# Autodesk Inventor assembly: Door 2
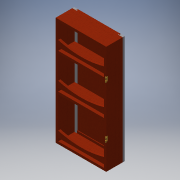
[picture p0: Inventor's stored thumbnail of the model, 180x180]
Saved by Autodesk Inventor 2016 (Build 200138000, 138)
## iProperties
Created: 2017-10-31
Part Number: Door 2
Document SubType Name: Assembly
Designer: mathaetaes
Author: mathaetaes
## Documents named in this file (7)
- E:\Projects\3D Printer\printer projects\My Designs\Bar Cabinet 2.20.2018\Door 2.iam
- E:\Projects\3D Printer\printer projects\My Designs\Bar Cabinet 2.20.2018\Door top.ipt
- E:\Projects\3D Printer\printer projects\My Designs\Bar Cabinet 2.20.2018\Door retention wall.ipt
- E:\Projects\3D Printer\printer projects\My Designs\Bar Cabinet 2.20.2018\Door Shelf.ipt
- E:\Projects\3D Printer\printer projects\My Designs\Bar Cabinet 2.20.2018\Door 2 Side.ipt
- E:\Projects\3D Printer\printer projects\My Designs\Bar Cabinet 2.20.2018\Door Moulding Assembled.iam
- E:\Projects\3D Printer\printer projects\My Designs\Bar Cabinet 2.20.2018\hinge left.ipt
## Components (12 placed, 6 different names)
1. Door top:1 — Flush:21, Flush:22, Mate:32, Flush:30, Flush:31, Mate:33, Flush:33
2. Door retention wall:1 — Mate:20, Flush:20, Mate:34
3. Door Shelf:1 — Mate:10, Mate:12, Mate:15, Flush:15, Flush:16, Mate:19
4. Door retention wall:2 — Mate:10, Flush:14, Mate:16
5. Door 2 Side:2 — Flush:14, Mate:12, Flush:15, Mate:16, Mate:19, Mate:20, Flush:20, Flush:21, Mate:22, Flush:26, Mate:29, Mate:31, Flush:28, Flush:29, Mate:32, Flush:30, Flush:31, Flush:32, Mate:35, Mate:36, Mate:37, Mate:38, Mate:39, Mate:40
6. Door 2 Side:3 — Mate:15, Flush:16, Flush:22, Mate:23, Mate:24, Flush:27, Mate:30
7. Door Shelf:3 — Mate:22, Mate:23, Mate:24, Flush:26, Mate:28
8. Door retention wall:4 — Mate:28, Flush:27, Mate:29, Mate:30
9. Door top:2 — Mate:31, Flush:28, Flush:29, Mate:34
10. Door Moulding Assembled:1 [sub-assembly] — Mate:33, Flush:32, Flush:33
11. hinge left:1 — Mate:35, Mate:37, Mate:38
12. hinge left:2 — Mate:36, Mate:39, Mate:40
## Relationships (36: Mate 22, Flush 14)
- Mate:10 (25.4 mm): Door Shelf:1 ↔ Door retention wall:2
- Flush:14: Door retention wall:2 ↔ Door 2 Side:2
- Mate:12: Door Shelf:1 ↔ Door 2 Side:2
- Mate:15: Door Shelf:1 ↔ Door 2 Side:3
- Flush:15: Door Shelf:1 ↔ Door 2 Side:2
- Mate:16: Door retention wall:2 ↔ Door 2 Side:2
- Flush:16: Door Shelf:1 ↔ Door 2 Side:3
- Mate:19: Door Shelf:1 ↔ Door 2 Side:2
- Mate:20: Door retention wall:1 ↔ Door 2 Side:2
- Flush:20: Door retention wall:1 ↔ Door 2 Side:2
- Flush:21: Door top:1 ↔ Door 2 Side:2
- Flush:22: Door top:1 ↔ Door 2 Side:3
- Mate:22: Door 2 Side:2 ↔ Door Shelf:3
- Mate:23: Door 2 Side:3 ↔ Door Shelf:3
- Mate:24: Door 2 Side:3 ↔ Door Shelf:3
- Flush:26: Door 2 Side:2 ↔ Door Shelf:3
- Mate:28 (25.4 mm): Door Shelf:3 ↔ Door retention wall:4
- Flush:27: Door 2 Side:3 ↔ Door retention wall:4
- Mate:29: Door 2 Side:2 ↔ Door retention wall:4
- Mate:30: Door 2 Side:3 ↔ Door retention wall:4
- Mate:31: Door 2 Side:2 ↔ Door top:2
- Flush:28: Door 2 Side:2 ↔ Door top:2
- Flush:29: Door 2 Side:2 ↔ Door top:2
- Mate:32: Door top:1 ↔ Door 2 Side:2
- Flush:30: Door top:1 ↔ Door 2 Side:2
- Flush:31: Door top:1 ↔ Door 2 Side:2
- Mate:33: Door top:1 ↔ Door Moulding Assembled:1
- Flush:32: Door 2 Side:2 ↔ Door Moulding Assembled:1
- Flush:33: Door top:1 ↔ Door Moulding Assembled:1
- Mate:34 (25.4 mm): Door retention wall:1 ↔ Door top:2
- Mate:35: Door 2 Side:2 ↔ hinge left:1
- Mate:36: Door 2 Side:2 ↔ hinge left:2
- Mate:37: Door 2 Side:2 ↔ hinge left:1
- Mate:38: Door 2 Side:2 ↔ hinge left:1
- Mate:39: Door 2 Side:2 ↔ hinge left:2
- Mate:40: Door 2 Side:2 ↔ hinge left:2
